# Autodesk Inventor assembly: ASSY_REV,ENG_DESIGN2
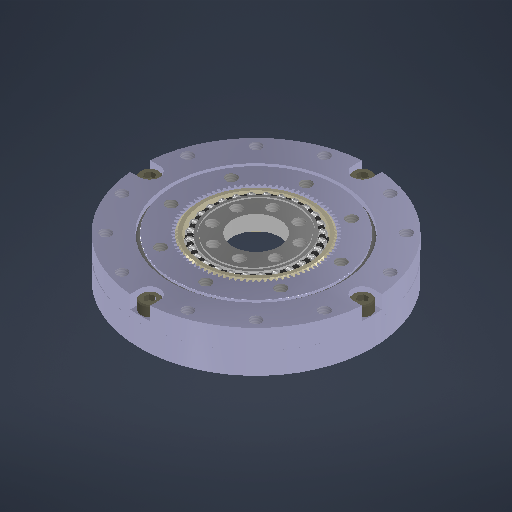
[picture p0: Inventor's stored thumbnail of the model, 512x512]
Saved by Autodesk Inventor 2026.2 (Build 302298010, 298A)
## iProperties
Created: 2026-02-10
Part Number: ASSY_REV,ENG_DESIGN2
Document SubType Name: Assembly
Designer: 4aida
Author: 4aida
## Documents named in this file (15)
- C:\Users\4aida\OneDrive\Documents\GitHub\Design_II_Group6\REV_ENG\ASSY_REV,ENG_DESIGN2.iam
- C:\Users\4aida\OneDrive\Documents\GitHub\Design_II_Group6\REV_ENG\ROLLER_CR_BEARING,REV-ENG.ipt
- C:\Users\4aida\OneDrive\Documents\GitHub\Design_II_Group6\REV_ENG\SPACER_ROLLER_CR_BEARING,REV-ENG.ipt
- C:\Users\4aida\OneDrive\Documents\GitHub\Design_II_Group6\REV_ENG\MIR_SPACER_ROLLER_CR_BEARING,REV-ENG.ipt
- C:\Users\4aida\OneDrive\Documents\GitHub\Design_II_Group6\REV_ENG\CR_ROLLER_BOUNDRY,REV-ENG.ipt
- C:\Users\4aida\OneDrive\Documents\GitHub\Design_II_Group6\REV_ENG\O_RING.ipt
- C:\Users\4aida\OneDrive\Documents\GitHub\Design_II_Group6\REV_ENG\CR_OUTSIDE,BOTTOM,REV-ENG.ipt
- C:\Users\4aida\OneDrive\Documents\GitHub\Design_II_Group6\REV_ENG\CR_OUTSIDE,TOP,REV-ENG.ipt
- C:\Users\4aida\OneDrive\Documents\GitHub\Design_II_Group6\REV_ENG\Fasteners\M3\SCREW,SOCKET-HD,P,12_9,M03X0_5X10MM.ipt
- C:\Users\4aida\OneDrive\Documents\GitHub\Design_II_Group6\REV_ENG\2.5mm_BALL_BEARINGS.ipt
- C:\Users\4aida\OneDrive\Documents\GitHub\Design_II_Group6\REV_ENG\Flex_SPLINE,REV-ENG.iam
- C:\Users\4aida\OneDrive\Documents\GitHub\Design_II_Group6\REV_ENG\DERIVEN_CR_INSIDE,REV-ENG.ipt
- C:\Users\4aida\OneDrive\Documents\GitHub\Design_II_Group6\REV_ENG\ELIPSE_DRIVE,REV-ENG.ipt
- C:\Users\4aida\OneDrive\Documents\GitHub\Design_II_Group6\REV_ENG\BOTTOM_ELIP_BEARING_SEAL,REV-ENG.ipt
- C:\Users\4aida\OneDrive\Documents\GitHub\Design_II_Group6\REV_ENG\DERIVEN_BALL_BEARING,REV-ENG.ipt
## Components (62 placed, 14 different names)
1. CR_ROLLER_BOUNDRY,REV-ENG:1 — Mate:23, Mate:24
2. O_RING:1 — Mate:16, Tangent:7
3. CR_OUTSIDE,BOTTOM,REV-ENG:1 — Mate:9, Mate:10, Mate:13, Flush:4, Mate:25, Mate:26
4. CR_OUTSIDE,TOP,REV-ENG:1 — Mate:9, Mate:10, Mate:12, Insert:1, Insert:2, Insert:3, Insert:4, Mate:27, Mate:28, Flush:8
5. SCREW,SOCKET-HD,P,12_9,M03X0_5X10MM:1 — Insert:1
6. Flex_SPLINE,REV-ENG:1 [sub-assembly] — Flush:5, Mate:15, Mate:25, Mate:16, Mate:29
7. DERIVEN_CR_INSIDE,REV-ENG:1 — Flush:5, Mate:15, Tangent:7, Mate:18, Mate:21, Tangent:8, Tangent:9, Mate:28, Flush:8, Flush:9, Rotation:1
8. SCREW,SOCKET-HD,P,12_9,M03X0_5X10MM:2 — Insert:4
9. SCREW,SOCKET-HD,P,12_9,M03X0_5X10MM:3 — Insert:2
10. SCREW,SOCKET-HD,P,12_9,M03X0_5X10MM:4 — Insert:3
11. ELIPSE_DRIVE,REV-ENG:1 — Flush:9, Tangent:10, Mate:31, Flush:10, Mate:33, Rotation:1, Mate:34, Mate:35, Mate:37
12. 2.5mm_BALL_BEARINGS:3 — Mate:30, Tangent:10, Mate:31, Mate:36
13. BOTTOM_ELIP_BEARING_SEAL,REV-ENG:1 — Mate:32, Flush:10, Mate:33
14. DERIVEN_BALL_BEARING,REV-ENG:1 — Mate:34, Mate:35, Mate:36
15. MIR_SPACER_ROLLER_CR_BEARING,REV-ENG:13 — Mate:21, Mate:22
16. ROLLER_CR_BEARING,REV-ENG:27 — Mate:20, Mate:22, Tangent:8
17. SPACER_ROLLER_CR_BEARING,REV-ENG:13 — Mate:18, Mate:19, Flush:7, Mate:20
18. ROLLER_CR_BEARING,REV-ENG:26 — Mate:19, Tangent:9
19. MIR_SPACER_ROLLER_CR_BEARING,REV-ENG:14
20. ROLLER_CR_BEARING,REV-ENG:28
21. SPACER_ROLLER_CR_BEARING,REV-ENG:14
22. ROLLER_CR_BEARING,REV-ENG:29
23. MIR_SPACER_ROLLER_CR_BEARING,REV-ENG:15
24. ROLLER_CR_BEARING,REV-ENG:30
25. SPACER_ROLLER_CR_BEARING,REV-ENG:15
26. ROLLER_CR_BEARING,REV-ENG:31
27. MIR_SPACER_ROLLER_CR_BEARING,REV-ENG:16
28. ROLLER_CR_BEARING,REV-ENG:32
29. SPACER_ROLLER_CR_BEARING,REV-ENG:16
30. ROLLER_CR_BEARING,REV-ENG:33
31. MIR_SPACER_ROLLER_CR_BEARING,REV-ENG:17
32. ROLLER_CR_BEARING,REV-ENG:34
33. SPACER_ROLLER_CR_BEARING,REV-ENG:17
34. ROLLER_CR_BEARING,REV-ENG:35
35. MIR_SPACER_ROLLER_CR_BEARING,REV-ENG:18
36. ROLLER_CR_BEARING,REV-ENG:36
37. SPACER_ROLLER_CR_BEARING,REV-ENG:18
38. ROLLER_CR_BEARING,REV-ENG:37
39. MIR_SPACER_ROLLER_CR_BEARING,REV-ENG:19
40. ROLLER_CR_BEARING,REV-ENG:38
41. SPACER_ROLLER_CR_BEARING,REV-ENG:19
42. ROLLER_CR_BEARING,REV-ENG:39
43. MIR_SPACER_ROLLER_CR_BEARING,REV-ENG:20
44. ROLLER_CR_BEARING,REV-ENG:40
45. SPACER_ROLLER_CR_BEARING,REV-ENG:20
46. ROLLER_CR_BEARING,REV-ENG:41
47. MIR_SPACER_ROLLER_CR_BEARING,REV-ENG:21
48. ROLLER_CR_BEARING,REV-ENG:42
49. SPACER_ROLLER_CR_BEARING,REV-ENG:21
50. ROLLER_CR_BEARING,REV-ENG:43
51. MIR_SPACER_ROLLER_CR_BEARING,REV-ENG:22
52. ROLLER_CR_BEARING,REV-ENG:44
53. SPACER_ROLLER_CR_BEARING,REV-ENG:22
54. ROLLER_CR_BEARING,REV-ENG:45
55. MIR_SPACER_ROLLER_CR_BEARING,REV-ENG:23
56. ROLLER_CR_BEARING,REV-ENG:46
57. SPACER_ROLLER_CR_BEARING,REV-ENG:23
58. ROLLER_CR_BEARING,REV-ENG:47
59. MIR_SPACER_ROLLER_CR_BEARING,REV-ENG:24
60. ROLLER_CR_BEARING,REV-ENG:48
61. SPACER_ROLLER_CR_BEARING,REV-ENG:24
62. ROLLER_CR_BEARING,REV-ENG:49
## Component patterns: (12 elements, first: MIR_SPACER_ROLLER_CR_BEARING,REV-ENG:13 + ROLLER_CR_BEARING,REV-ENG:27 + SPACER_ROLLER_CR_BEARING,REV-ENG:13 + ROLLER_CR_BEARING,REV-ENG:26)
## Relationships (41: Mate 26, Flush 6, Tangent 4, Insert 4, RelateRotation 1)
- Mate:9: CR_OUTSIDE,BOTTOM,REV-ENG:1 ↔ CR_OUTSIDE,TOP,REV-ENG:1
- Mate:10: CR_OUTSIDE,BOTTOM,REV-ENG:1 ↔ CR_OUTSIDE,TOP,REV-ENG:1
- Mate:12: CR_OUTSIDE,TOP,REV-ENG:1
- Mate:13: CR_OUTSIDE,BOTTOM,REV-ENG:1
- Flush:4: CR_OUTSIDE,BOTTOM,REV-ENG:1
- Flush:5: Flex_SPLINE,REV-ENG:1 ↔ DERIVEN_CR_INSIDE,REV-ENG:1
- Mate:15: Flex_SPLINE,REV-ENG:1 ↔ DERIVEN_CR_INSIDE,REV-ENG:1
- Mate:16: O_RING:1 ↔ Flex_SPLINE,REV-ENG:1
- Tangent:7: O_RING:1 ↔ DERIVEN_CR_INSIDE,REV-ENG:1
- Mate:18: DERIVEN_CR_INSIDE,REV-ENG:1 ↔ SPACER_ROLLER_CR_BEARING,REV-ENG:13
- Mate:19: SPACER_ROLLER_CR_BEARING,REV-ENG:13 ↔ ROLLER_CR_BEARING,REV-ENG:26
- Flush:7: SPACER_ROLLER_CR_BEARING,REV-ENG:13
- Mate:20: ROLLER_CR_BEARING,REV-ENG:27 ↔ SPACER_ROLLER_CR_BEARING,REV-ENG:13
- Mate:21: DERIVEN_CR_INSIDE,REV-ENG:1 ↔ MIR_SPACER_ROLLER_CR_BEARING,REV-ENG:13
- Mate:22: MIR_SPACER_ROLLER_CR_BEARING,REV-ENG:13 ↔ ROLLER_CR_BEARING,REV-ENG:27
- Tangent:8 (0.125 mm): DERIVEN_CR_INSIDE,REV-ENG:1 ↔ ROLLER_CR_BEARING,REV-ENG:27
- Tangent:9 (0.125 mm): DERIVEN_CR_INSIDE,REV-ENG:1 ↔ ROLLER_CR_BEARING,REV-ENG:26
- Mate:23: CR_ROLLER_BOUNDRY,REV-ENG:1
- Mate:24: CR_ROLLER_BOUNDRY,REV-ENG:1
- Mate:25: CR_OUTSIDE,BOTTOM,REV-ENG:1 ↔ Flex_SPLINE,REV-ENG:1
- Insert:1: CR_OUTSIDE,TOP,REV-ENG:1 ↔ SCREW,SOCKET-HD,P,12_9,M03X0_5X10MM:1
- Insert:2: CR_OUTSIDE,TOP,REV-ENG:1 ↔ SCREW,SOCKET-HD,P,12_9,M03X0_5X10MM:3
- Insert:3: CR_OUTSIDE,TOP,REV-ENG:1 ↔ SCREW,SOCKET-HD,P,12_9,M03X0_5X10MM:4
- Insert:4: CR_OUTSIDE,TOP,REV-ENG:1 ↔ SCREW,SOCKET-HD,P,12_9,M03X0_5X10MM:2
- Mate:26: CR_OUTSIDE,BOTTOM,REV-ENG:1
- Mate:27: CR_OUTSIDE,TOP,REV-ENG:1
- Mate:28: CR_OUTSIDE,TOP,REV-ENG:1 ↔ DERIVEN_CR_INSIDE,REV-ENG:1
- Flush:8: CR_OUTSIDE,TOP,REV-ENG:1 ↔ DERIVEN_CR_INSIDE,REV-ENG:1
- Flush:9: DERIVEN_CR_INSIDE,REV-ENG:1 ↔ ELIPSE_DRIVE,REV-ENG:1
- Mate:29: Flex_SPLINE,REV-ENG:1
- Mate:30: 2.5mm_BALL_BEARINGS:3
- Tangent:10: ELIPSE_DRIVE,REV-ENG:1 ↔ 2.5mm_BALL_BEARINGS:3
- Mate:31: ELIPSE_DRIVE,REV-ENG:1 ↔ 2.5mm_BALL_BEARINGS:3
- Mate:32: BOTTOM_ELIP_BEARING_SEAL,REV-ENG:1
- Flush:10 (0.375 mm): ELIPSE_DRIVE,REV-ENG:1 ↔ BOTTOM_ELIP_BEARING_SEAL,REV-ENG:1
- Mate:33: ELIPSE_DRIVE,REV-ENG:1 ↔ BOTTOM_ELIP_BEARING_SEAL,REV-ENG:1
- Rotation:1 [RelateRotation] (0.0116 ul): DERIVEN_CR_INSIDE,REV-ENG:1 ↔ ELIPSE_DRIVE,REV-ENG:1
- Mate:34: ELIPSE_DRIVE,REV-ENG:1 ↔ DERIVEN_BALL_BEARING,REV-ENG:1
- Mate:35: ELIPSE_DRIVE,REV-ENG:1 ↔ DERIVEN_BALL_BEARING,REV-ENG:1
- Mate:36: 2.5mm_BALL_BEARINGS:3 ↔ DERIVEN_BALL_BEARING,REV-ENG:1
- Mate:37: ELIPSE_DRIVE,REV-ENG:1
